# Autodesk Inventor assembly: hf23sp_0
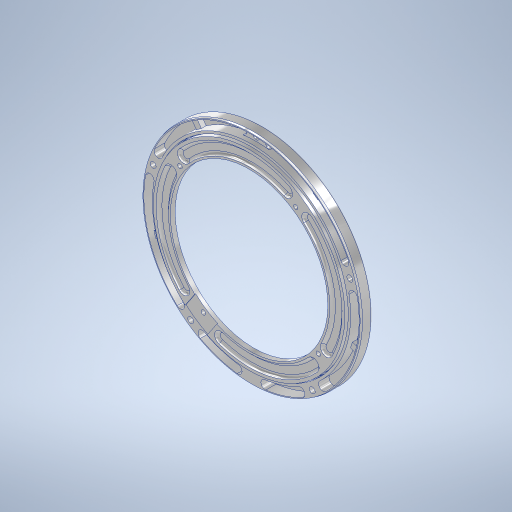
[picture p0: Inventor's stored thumbnail of the model, 512x512]
Saved by Autodesk Inventor 2024 (Build 280153000, 153)
## iProperties
Created: 2015-07-06
Part Number: hf23sp_0
Description: STEP AP203
Document SubType Name: Assembly
Designer: Hagihara Yuya
Mass: 370 g
Surface Area: 876.645 cm^2
Volume: 97.9505 cm^3
Density: 3.77742 g/cm^3
Sending System: SolidWorks 2012
Preprocessor: SwSTEP 2.0
Title: SC210-11538_HF23SP_^[e[u_0.step
Revision Number: ANY
## Documents named in this file (3)
- C:\Users\田之上巧太\Documents\Inventor\キャチロボ2024\BasicParts\TurnTable\hf23sp_0\hf23sp_0.iam
- C:\Users\田之上巧太\Documents\Inventor\キャチロボ2024\BasicParts\TurnTable\hf23sp_0\SC210-11534_HF23SP_x_[Xv_[g.ipt
- C:\Users\田之上巧太\Documents\Inventor\キャチロボ2024\BasicParts\TurnTable\hf23sp_0\SC210-11535_HF23SP_gbvv_[g.ipt
## Components (2 placed, 2 different names)
1. SC210-11534_HF23SP_x[Xv[g_1 — 回転:1
2. SC210-11535_HF23SP_gbvv[g_2 — 回転:1
## Relationships (1: RevoluteJoint 1)
- 回転:1 [RevoluteJoint] (-4.5 mm): SC210-11534_HF23SP_x[Xv[g_1 ↔ SC210-11535_HF23SP_gbvv[g_2
